# Autodesk Inventor assembly: plates
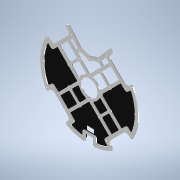
[picture p0: Inventor's stored thumbnail of the model, 180x180]
Saved by Autodesk Inventor 2020 (Build 240168000, 168)
## iProperties
Created: 2024-03-27
Part Number: plates
Document SubType Name: Assembly
Designer: 4s
Author: 4s
## Documents named in this file (3)
- C:\Users\4s\Documents\Inventor models\Asterisk\plates.iam
- C:\Users\4s\Documents\Inventor models\Asterisk\robot_v2\upper_plate.ipt
- C:\Users\4s\Documents\Altium projects\Asterisk Main Board\Main board 3d\Board.iam
## Components (2 placed, 2 different names)
1. upper_plate:1 — Совмещение:1, Совмещение:2, Заподлицо:1, Совмещение:3, Совмещение:4, Совмещение:5
2. Board:1 [sub-assembly] — Совмещение:3, Совмещение:4, Совмещение:5
## Relationships (6: Mate 5, Flush 1)
- Совмещение:1 [Mate]: upper_plate:1
- Совмещение:2 [Mate]: upper_plate:1
- Заподлицо:1 [Flush]: upper_plate:1
- Совмещение:3 [Mate]: upper_plate:1 ↔ Board:1
- Совмещение:4 [Mate]: upper_plate:1 ↔ Board:1
- Совмещение:5 [Mate]: upper_plate:1 ↔ Board:1
